# Autodesk Inventor assembly: Hybrid
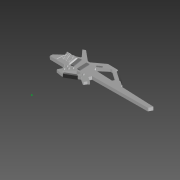
[picture p0: Inventor's stored thumbnail of the model, 180x180]
Saved by Autodesk Inventor 2020.4 (Build 244396010, 396A)
## iProperties
Created: 2022-11-11
Part Number: Hybrid
Document SubType Name: Assembly
Designer: valer
Author: valer
## Documents named in this file (7)
- C:\Users\Val\Desktop\hybrid\src\Hybrid.iam
- C:\Users\Val\Desktop\hybrid\src\Hybrid.ipt
- C:\Users\Val\Desktop\hybrid\src\OscilloscopeScreen.ipt
- C:\Users\Val\Desktop\hybrid\src\BottomGrip.ipt
- C:\Users\Val\Desktop\hybrid\src\TopGrip.ipt
- C:\Users\Val\Desktop\hybrid\src\BassTuner.ipt
- C:\Users\Val\Desktop\hybrid\src\MidiPickup.ipt
## Components (10 placed, 6 different names)
1. Hybrid:1 — Flush:2, Mate:2, Mate:3, Mate:13, Mate:14, Mate:15
2. OscilloscopeScreen:1 — Flush:2, Mate:2, Mate:3
3. BottomGrip:1 — Mate:14, Mate:15
4. TopGrip:1
5. BassTuner:1
6. BassTuner:2
7. BassTuner:3
8. BassTuner:4
9. BassTuner:5
10. MidiPickup:1 — Mate:13
## Relationships (6: Mate 5, Flush 1)
- Flush:2: Hybrid:1 ↔ OscilloscopeScreen:1
- Mate:2: Hybrid:1 ↔ OscilloscopeScreen:1
- Mate:3: Hybrid:1 ↔ OscilloscopeScreen:1
- Mate:13: Hybrid:1 ↔ MidiPickup:1
- Mate:14: Hybrid:1 ↔ BottomGrip:1
- Mate:15: Hybrid:1 ↔ BottomGrip:1
